# Autodesk Inventor assembly: nut bolt practise
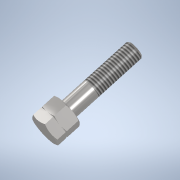
[picture p0: Inventor's stored thumbnail of the model, 180x180]
Saved by Autodesk Inventor 2022 (Build 260153000, 153)
## iProperties
Created: 2022-03-12
Part Number: nut bolt practise
Document SubType Name: Assembly
Designer: karee
Author: karee
## Documents named in this file (3)
- C:\Users\karee\OneDrive\Desktop\nut bolt practise.iam
- C:\Users\karee\OneDrive\Documents\Inventor\Content Center Files\R2022\en-US\PN-85 M-82101 A\PN-85_M-82101 - M 8 x 40 - 1.25(1).ipt
- C:\Users\karee\OneDrive\Documents\Inventor\Content Center Files\R2022\en-US\ANSI B 18.2.4.1 M(1)\ANSI B 18.2.4.1 M - M8 x 1.25Style 1.ipt
## Components (2 placed, 2 different names)
1. PN-85/M-82101 Product grade A M 8 x 40:1 — Mate:1, Mate:2
2. Hex Nut Metric M8 x 1.25:1 — Mate:1, Mate:2
## Relationships (2: Mate 2)
- Mate:1: PN-85/M-82101 Product grade A M 8 x 40:1 ↔ Hex Nut Metric M8 x 1.25:1
- Mate:2: PN-85/M-82101 Product grade A M 8 x 40:1 ↔ Hex Nut Metric M8 x 1.25:1
